# Autodesk Inventor assembly: AxisZ
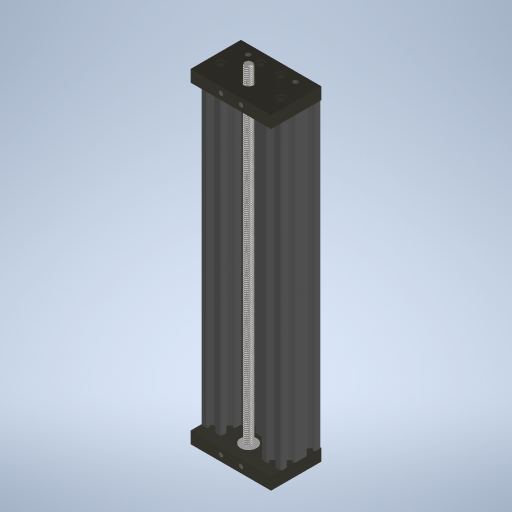
[picture p0: Inventor's stored thumbnail of the model, 512x512]
Saved by Autodesk Inventor 2024.2 (Build 282272000, 272)
## iProperties
Created: 2024-08-27
Part Number: AxisZ
Document SubType Name: Assembly
Designer: Admin
Author: Admin
## Documents named in this file (5)
- C:\Users\Admin\Documents\GitHub\RobotCartesiano\DiseñoBrazo\Assemblies\AxisZ.iam
- C:\Users\Admin\Documents\GitHub\RobotCartesiano\DiseñoBrazo\AluminumProfiles\AxisZ\LinearActuator\C-Beam4080.ipt
- C:\Users\Admin\Documents\GitHub\RobotCartesiano\DiseñoBrazo\AluminumProfiles\AxisZ\LinearActuator\C-BeamEnd.ipt
- C:\Users\Admin\Documents\GitHub\RobotCartesiano\DiseñoBrazo\AluminumProfiles\AxisZ\LinearActuator\Bearing8x16x5.ipt
- C:\Users\Admin\Documents\GitHub\RobotCartesiano\DiseñoBrazo\AluminumProfiles\AxisZ\LinearActuator\BallScrew.ipt
## Components (6 placed, 4 different names)
1. C-Beam4080:1 — Flush:1, Mate:1, Mate:2, Flush:2, Flush:3, Flush:4
2. C-BeamEnd:2 — Mate:2, Flush:3, Flush:4, Mate:3, Mate:4, Flush:5
3. C-BeamEnd:3 — Flush:1, Mate:1, Flush:2, Mate:5, Mate:6, Mate:7
4. Bearing8x16x5:1 — Mate:3, Mate:4
5. Bearing8x16x5:2 — Mate:5, Mate:6
6. BallScrew:1 — Mate:7, Flush:5
## Relationships (12: Mate 7, Flush 5)
- Flush:1: C-Beam4080:1 ↔ C-BeamEnd:3
- Mate:1: C-Beam4080:1 ↔ C-BeamEnd:3
- Mate:2: C-Beam4080:1 ↔ C-BeamEnd:2
- Flush:2: C-Beam4080:1 ↔ C-BeamEnd:3
- Flush:3: C-Beam4080:1 ↔ C-BeamEnd:2
- Flush:4: C-Beam4080:1 ↔ C-BeamEnd:2
- Mate:3: C-BeamEnd:2 ↔ Bearing8x16x5:1
- Mate:4: C-BeamEnd:2 ↔ Bearing8x16x5:1
- Mate:5: C-BeamEnd:3 ↔ Bearing8x16x5:2
- Mate:6: C-BeamEnd:3 ↔ Bearing8x16x5:2
- Mate:7: C-BeamEnd:3 ↔ BallScrew:1
- Flush:5: C-BeamEnd:2 ↔ BallScrew:1
